# Autodesk Inventor assembly: Bend Piece 1764
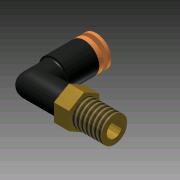
[picture p0: Inventor's stored thumbnail of the model, 180x180]
Saved by Autodesk Inventor 2011 (Build 150239000, 239)
## iProperties
Created: 2010-02-15
Part Number: Bend Piece 1764
Document SubType Name: Assembly
Designer: jgehrig
Author: jgehrig
## Documents named in this file (4)
- R:\CAD Archives\Pnewmatics\Pnematics Bend Piece\Bend Piece 1764.iam
- R:\CAD Archives\Pnewmatics\Pnematics Bend Piece\Bend Piece.ipt
- R:\CAD Archives\Pnewmatics\Pnematics Bend Piece\pnematic screw part .ipt
- R:\CAD Archives\Pnewmatics\pnewmatic screw\pnematic screw part 2.ipt
## Components (3 placed, 3 different names)
1. Bend Piece:1 — Insert:1, Insert:2
2. pnematic screw part :1 — Insert:2
3. pnematic screw part 2:1 — Insert:1
## Relationships (2: Insert 2)
- Insert:1: Bend Piece:1 ↔ pnematic screw part 2:1
- Insert:2: Bend Piece:1 ↔ pnematic screw part :1
